# Autodesk Inventor assembly: claws_endeffector_3
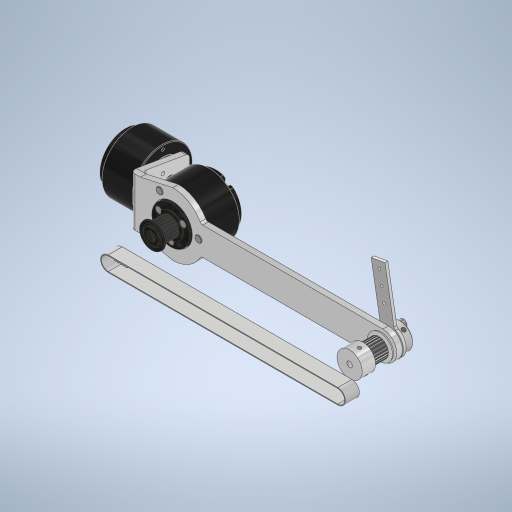
[picture p0: Inventor's stored thumbnail of the model, 512x512]
Saved by Autodesk Inventor 2024 (Build 280153000, 153)
## iProperties
Created: 2025-03-10
Part Number: claws_endeffector_3
Document SubType Name: Assembly
Designer: 1412z
Author: 1412z
## Documents named in this file (13)
- C:\Users\1412z\OneDrive\デスクトップ\rdclab\harvesting_robot\harvesting_endeffector\claws_endeffector\claws_endeffector_3.iam
- C:\Users\1412z\OneDrive\デスクトップ\rdclab\harvesting_robot\harvesting_endeffector\claws_endeffector\motor_holder\motor_holder_3.ipt
- C:\Users\1412z\OneDrive\デスクトップ\rdclab\harvesting_robot\harvesting_endeffector\claws_endeffector\GIM3505-08\GIM3505-8_with-driver.ipt
- C:\Users\1412z\OneDrive\デスクトップ\rdclab\harvesting_robot\harvesting_endeffector\claws_endeffector\misumi\HTPA22S2M100-A-V4-Z6-J3_Autodesk_Inventor_2024_20250304\HTPA22S2M100-A-V4-Z6-J3_0_a.ipt
- C:\Users\1412z\OneDrive\デスクトップ\rdclab\harvesting_robot\harvesting_endeffector\claws_endeffector\misumi\M2.5×4\M2.5×4.ipt
- C:\Users\1412z\OneDrive\デスクトップ\rdclab\harvesting_robot\harvesting_endeffector\claws_endeffector\misumi\SFL674ZZ_Autodesk_Inventor_2024_20250304\SFL674ZZ.ipt
- C:\Users\1412z\OneDrive\デスクトップ\rdclab\harvesting_robot\harvesting_endeffector\claws_endeffector\misumi\simring\simring_Φ4-Φ5.ipt
- C:\Users\1412z\OneDrive\デスクトップ\rdclab\harvesting_robot\harvesting_endeffector\claws_endeffector\misumi\HTPA22S2M100-K-P4_Autodesk_Inventor_2024_20250304\AIS2024\HTPA22S2M100-K-P4_a.ipt
- C:\Users\1412z\OneDrive\デスクトップ\rdclab\harvesting_robot\harvesting_endeffector\claws_endeffector\misumi\HTBN360S2M-100_Autodesk_Inventor_2024_20250304\HTBN360S2M-100_info-1-16-16.ipt
- C:\Users\1412z\OneDrive\デスクトップ\rdclab\harvesting_robot\harvesting_endeffector\claws_endeffector\cutter_part\cutter_board.ipt
- C:\Users\1412z\OneDrive\デスクトップ\rdclab\harvesting_robot\harvesting_endeffector\claws_endeffector\misumi\SSCMN4_Autodesk_Inventor_2024_20250310\AIS2024\SSCMN4b.ipt
- C:\Users\1412z\OneDrive\デスクトップ\rdclab\harvesting_robot\harvesting_endeffector\claws_endeffector\misumi\M3×8\M3×8.ipt
- C:\Users\1412z\OneDrive\デスクトップ\rdclab\harvesting_robot\harvesting_endeffector\claws_endeffector\misumi\shaft\shaft.ipt
## Components (21 placed, 12 different names)
1. motor_holder_3:1 — 回転:1, 回転:2, 回転:3, 回転:4, 回転:10, 回転:11, 回転:21, 回転:22, 回転:23
2. GIM3505-8_with-driver:1 — 回転:1, 回転:2, 回転:5, 回転:6
3. GIM3505-8_with-driver:2 — 回転:3, 回転:4
4. HTPA22S2M100-A-V4-Z6-J3_0_a:1 — 回転:5, 回転:6, 回転:7, 回転:8, 回転:9
5. M2.5×4:1 — 回転:8
6. M2.5×4:2 — 回転:7
7. M2.5×4:3 — 回転:9
8. SFL674ZZ:1 — 回転:10, 回転:12
9. SFL674ZZ:2 — 回転:11, 回転:13
10. simring_Φ4-Φ5:1 — 回転:13, 回転:14
11. simring_Φ4-Φ5:2 — 回転:12, 回転:15
12. HTPA22S2M100-K-P4_a:1 — 回転:14, 回転:20
13. HTBN360S2M-100_info-1-16-16:1
14. cutter_board:1 — 回転:15, 回転:16, 回転:17
15. SSCMN4b:1 — 回転:16, 回転:17, 回転:18, 回転:19
16. M3×8:1 — 回転:18
17. M3×8:2 — 回転:19
18. shaft:1 — 回転:20
19. M2.5×4:4 — 回転:23
20. M2.5×4:5 — 回転:22
21. M2.5×4:6 — 回転:21
## Relationships (23: RevoluteJoint 23)
- 回転:1 [RevoluteJoint]: motor_holder_3:1 ↔ GIM3505-8_with-driver:1
- 回転:2 [RevoluteJoint]: motor_holder_3:1 ↔ GIM3505-8_with-driver:1
- 回転:3 [RevoluteJoint]: motor_holder_3:1 ↔ GIM3505-8_with-driver:2
- 回転:4 [RevoluteJoint]: motor_holder_3:1 ↔ GIM3505-8_with-driver:2
- 回転:5 [RevoluteJoint]: GIM3505-8_with-driver:1 ↔ HTPA22S2M100-A-V4-Z6-J3_0_a:1
- 回転:6 [RevoluteJoint]: GIM3505-8_with-driver:1 ↔ HTPA22S2M100-A-V4-Z6-J3_0_a:1
- 回転:7 [RevoluteJoint]: HTPA22S2M100-A-V4-Z6-J3_0_a:1 ↔ M2.5×4:2
- 回転:8 [RevoluteJoint]: HTPA22S2M100-A-V4-Z6-J3_0_a:1 ↔ M2.5×4:1
- 回転:9 [RevoluteJoint]: HTPA22S2M100-A-V4-Z6-J3_0_a:1 ↔ M2.5×4:3
- 回転:10 [RevoluteJoint]: motor_holder_3:1 ↔ SFL674ZZ:1
- 回転:11 [RevoluteJoint]: motor_holder_3:1 ↔ SFL674ZZ:2
- 回転:12 [RevoluteJoint]: SFL674ZZ:1 ↔ simring_Φ4-Φ5:2
- 回転:13 [RevoluteJoint]: SFL674ZZ:2 ↔ simring_Φ4-Φ5:1
- 回転:14 [RevoluteJoint]: simring_Φ4-Φ5:1 ↔ HTPA22S2M100-K-P4_a:1
- 回転:15 [RevoluteJoint]: simring_Φ4-Φ5:2 ↔ cutter_board:1
- 回転:16 [RevoluteJoint]: cutter_board:1 ↔ SSCMN4b:1
- 回転:17 [RevoluteJoint]: cutter_board:1 ↔ SSCMN4b:1
- 回転:18 [RevoluteJoint]: SSCMN4b:1 ↔ M3×8:1
- 回転:19 [RevoluteJoint]: SSCMN4b:1 ↔ M3×8:2
- 回転:20 [RevoluteJoint]: HTPA22S2M100-K-P4_a:1 ↔ shaft:1
- 回転:21 [RevoluteJoint]: motor_holder_3:1 ↔ M2.5×4:6
- 回転:22 [RevoluteJoint]: motor_holder_3:1 ↔ M2.5×4:5
- 回転:23 [RevoluteJoint]: motor_holder_3:1 ↔ M2.5×4:4
